# Autodesk Inventor assembly: componentes
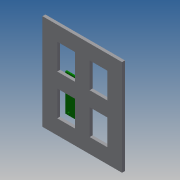
[picture p0: Inventor's stored thumbnail of the model, 180x180]
Saved by Autodesk Inventor 2017 (Build 210142000, 142)
## iProperties
Part Number: componentes
Material: Genérico
Document SubType Name: Assembly
Designer: FABLAB
Author: FABLAB
## Documents named in this file (3)
- C:\Users\FABLAB\Documents\GitHub\actor-re-actor\models\inventor-caja\Piezas\componentes.iam
- C:\Users\FABLAB\Documents\GitHub\actor-re-actor\models\inventor-caja\Case\bandeja componentes.ipt
- C:\Users\FABLAB\Documents\GitHub\actor-re-actor\models\inventor-caja\Piezas\driver motor.ipt
## Components (2 placed, 2 different names)
1. bandeja componentes:1 — Coincidencia:1, Nivelación:1, Nivelación:2
2. driver motor:1 — Coincidencia:1, Nivelación:1, Nivelación:2
## Relationships (3: Flush 2, Mate 1)
- Coincidencia:1 [Mate] (15 mm): bandeja componentes:1 ↔ driver motor:1
- Nivelación:1 [Flush] (12 mm): bandeja componentes:1 ↔ driver motor:1
- Nivelación:2 [Flush] (12 mm): bandeja componentes:1 ↔ driver motor:1
